# Autodesk Inventor assembly: LED Bacon
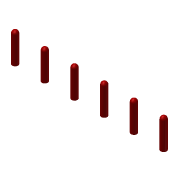
[picture p0: Inventor's stored thumbnail of the model, 180x180]
Saved by Autodesk Inventor 2015 (Build 190159000, 159)
## iProperties
Created: 2015-04-12
Part Number: LED Bacon
Document SubType Name: Assembly
Designer: Vukica
Author: Vukica
## Documents named in this file (2)
- C:\Users\Vukica\Dropbox\IEEE\hardware rules\2016Hardware_Court_v6\LED Bacon.iam
- C:\Users\Vukica\Dropbox\IEEE\hardware rules\2016Hardware_Court_v6\Beacon LED.ipt
## Components (6 placed, 1 different names)
1. Beacon LED:1 — Flush:1, Mate:1, Mate:3, Mate:5, Angle:1, Tangent:1
2. Beacon LED:2 — Flush:1, Flush:2, Mate:1, Mate:2, Tangent:4
3. Beacon LED:3 — Flush:2, Mate:2, Mate:3, Tangent:5, Mate:7, Flush:6
4. Beacon LED:4 — Mate:7, Flush:6
5. Beacon LED:5 — Flush:5, Mate:6, Tangent:3
6. Beacon LED:6 — Flush:5, Mate:5, Mate:6, Tangent:2
## Relationships (16: Mate 6, Tangent 5, Flush 4, Angle 1)
- Flush:1: Beacon LED:1 ↔ Beacon LED:2
- Flush:2: Beacon LED:2 ↔ Beacon LED:3
- Flush:5: Beacon LED:5 ↔ Beacon LED:6
- Mate:1 (25.4 mm): Beacon LED:1 ↔ Beacon LED:2
- Mate:2 (25.4 mm): Beacon LED:2 ↔ Beacon LED:3
- Mate:3 (50.8 mm): Beacon LED:1 ↔ Beacon LED:3
- Mate:5 (25.4 mm): Beacon LED:1 ↔ Beacon LED:6
- Mate:6 (25.4 mm): Beacon LED:5 ↔ Beacon LED:6
- Angle:1 (0 deg): Beacon LED:1
- Tangent:1: Beacon LED:1
- Tangent:2: Beacon LED:6
- Tangent:3: Beacon LED:5
- Tangent:4: Beacon LED:2
- Tangent:5: Beacon LED:3
- Mate:7 (25.4 mm): Beacon LED:3 ↔ Beacon LED:4
- Flush:6: Beacon LED:3 ↔ Beacon LED:4
